# Autodesk Inventor assembly: v1_rev4 1
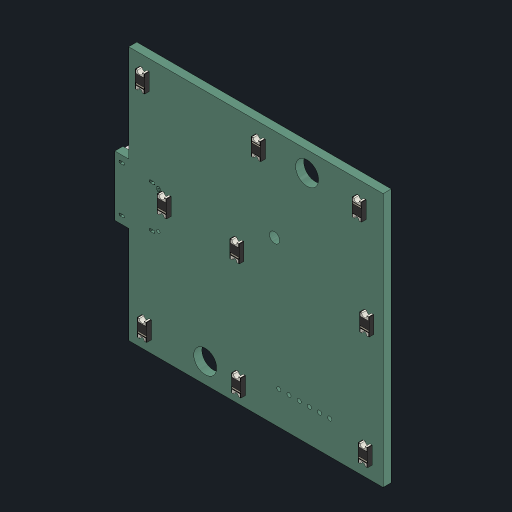
[picture p0: Inventor's stored thumbnail of the model, 512x512]
Saved by Autodesk Inventor 2023 (Build 270158000, 158)
## iProperties
Company: Kicad
Created: 2023-11-22
Part Number: v1_rev4 1
Description: KiCad electronic assembly
Document SubType Name: Assembly
Designer: leon.hergesic.adamov
Authority: Unknown
Sending System: KiCad to STEP converter
Preprocessor: Open CASCADE STEP processor 7.7
Title: v1_rev4.step
Author: Pcbnew
## Documents named in this file (8)
- C:\Users\Leon.hergesic.adamov\OneDrive\projekti_2022\24-lampadine\12-pcb\v1\export for inventor\v1-rev4\v1_rev4_exported.iam
- C:\Users\Leon.hergesic.adamov\OneDrive\projekti_2022\24-lampadine\12-pcb\v1\export for inventor\v1-rev4\D_1206_3216Metric.iam
- C:\Users\Leon.hergesic.adamov\OneDrive\projekti_2022\24-lampadine\12-pcb\v1\export for inventor\v1-rev4\SuperSOT-3.iam
- C:\Users\Leon.hergesic.adamov\OneDrive\projekti_2022\24-lampadine\12-pcb\v1\export for inventor\v1-rev4\C_1206_3216Metric.iam
- C:\Users\Leon.hergesic.adamov\OneDrive\projekti_2022\24-lampadine\12-pcb\v1\export for inventor\v1-rev4\R_0603_1608Metric.iam
- C:\Users\Leon.hergesic.adamov\OneDrive\projekti_2022\24-lampadine\12-pcb\v1\export for inventor\v1-rev4\SOT-223.iam
- C:\Users\Leon.hergesic.adamov\OneDrive\projekti_2022\24-lampadine\12-pcb\v1\export for inventor\v1-rev4\v1 PCB.ipt
- C:\Users\Leon.hergesic.adamov\OneDrive\projekti_2022\24-lampadine\99-foreign parts\usb_c_12401610E4#2A.ipt
## Components (29 placed, 29 different names)
1. 2 [sub-assembly]
2. 3 [sub-assembly]
3. 4 [sub-assembly]
4. 5 [sub-assembly]
5. 6 [sub-assembly]
6. 7 [sub-assembly]
7. 8 [sub-assembly]
8. 9 [sub-assembly]
9. 10 [sub-assembly]
10. 12 [sub-assembly]
11. 14 [sub-assembly]
12. 16 [sub-assembly]
13. 17 [sub-assembly]
14. 18 [sub-assembly]
15. 19 [sub-assembly]
16. 20 [sub-assembly]
17. 22 [sub-assembly]
18. 23 [sub-assembly]
19. 24 [sub-assembly]
20. 25 [sub-assembly]
21. 26 [sub-assembly]
22. 27 [sub-assembly]
23. 28 [sub-assembly]
24. 29 [sub-assembly]
25. 30 [sub-assembly]
26. 31 [sub-assembly]
27. 32 [sub-assembly]
28. 33 — Rigid:1
29. usb_c_12401610E4#2A:1 — Rigid:1
## Relationships (1: WeldJoint 1)
- Rigid:1 [WeldJoint]: 33 ↔ usb_c_12401610E4#2A:1
